# Autodesk Inventor assembly: Shoulder Joint Assembly
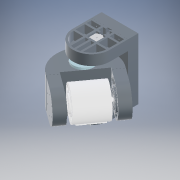
[picture p0: Inventor's stored thumbnail of the model, 180x180]
Saved by Autodesk Inventor 2017 SP1 (Build 210196100, 196)
## iProperties
Created: 2017-06-01
Part Number: Shoulder Joint Assembly
Document SubType Name: Assembly
Designer: Zach
Author: Zach
## Documents named in this file (15)
- C:\Users\Zach\Documents\GitHub\cr-laundry-robot\src\Body\Arm Assembly\Shoulder Joint Assembly\Shoulder Joint Assembly.iam
- C:\Users\Zach\Documents\GitHub\cr-laundry-robot\src\Body\Arm Assembly\Shoulder Joint Assembly\SJ002.ipt
- C:\Users\Zach\Documents\GitHub\cr-laundry-robot\src\Body\Arm Assembly\Shoulder Joint Assembly\SJ003.ipt
- C:\Users\Zach\Documents\GitHub\cr-laundry-robot\src\Body\Arm Assembly\Shoulder Joint Assembly\MC001.ipt
- C:\Users\Zach\Documents\GitHub\cr-laundry-robot\src\Body\Arm Assembly\Shoulder Joint Assembly\SJ001.ipt
- C:\Users\Zach\Documents\GitHub\cr-laundry-robot\src\Body\Arm Assembly\Shoulder Joint Assembly\MC002.ipt
- C:\Users\Zach\Documents\GitHub\cr-laundry-robot\lib\Stepper Motor - NEMA 17\NEMA17.ipt
- C:\Users\Zach\Documents\GitHub\cr-laundry-robot\src\Body\Arm Assembly\Shoulder Joint Assembly\SJ004.ipt
- C:\Users\Zach\Documents\GitHub\cr-laundry-robot\src\Body\Arm Assembly\Shoulder Joint Assembly\SJ005.ipt
- C:\Users\Zach\Documents\GitHub\cr-laundry-robot\src\Body\Arm Assembly\Shoulder Joint Assembly\SJ006.ipt
- C:\Users\Zach\Documents\GitHub\cr-laundry-robot\lib\U51105\U51105.ipt
- C:\Users\Zach\Documents\GitHub\cr-laundry-robot\lib\QS12MM250\QS12MM250.ipt
- C:\Users\Zach\Documents\GitHub\cr-laundry-robot\lib\6201RS\6201RS.ipt
- C:\Users\Zach\Documents\GitHub\cr-laundry-robot\src\Body\Arm Assembly\Shoulder Joint Assembly\SJ007.ipt
- C:\Users\Zach\Documents\GitHub\cr-laundry-robot\src\Body\Arm Assembly\Shoulder Joint Assembly\SJ008.ipt
## Components (29 placed, 14 different names)
1. MC001:1 — Mate:5, Mate:6, Mate:7, Mate:27, Mate:32
2. MC001:2 — Mate:41, Mate:42
3. SJ002:1 — Mate:1, Mate:4, Mate:5, Mate:6, Mate:7, Mate:8, Mate:9
4. SJ002:2 — Mate:18, Mate:19, Mate:20
5. SJ003:1 — Mate:1, Mate:4, Mate:8, Mate:9, Mate:18, Mate:19, Mate:20, Mate:71, Mate:72, Mate:73
6. SJ001:1 — Mate:23, Mate:24, Mate:25, Mate:43, Mate:44, Mate:47, Mate:48, Mate:49
7. MC002:1 — Mate:23, Mate:24, Mate:25, Mate:27, Mate:28, Mate:29, Mate:30, Mate:31
8. NEMA17:1 — Mate:28, Mate:29, Mate:30, Mate:31, Mate:32
9. SJ001:2 — Mate:37, Mate:38, Mate:39, Mate:43, Mate:45, Mate:46
10. MC002:2 — Mate:33, Mate:35, Mate:37, Mate:38, Mate:39, Mate:40, Mate:41
11. NEMA17:2 — Mate:33, Mate:35, Mate:40, Mate:42
12. SJ004:1 — Mate:44, Mate:45, Mate:46, Mate:57, Mate:58, Mate:59
13. SJ004:2 — Mate:47, Mate:48, Mate:49, Mate:54, Mate:55, Mate:56
14. SJ005:1 — Mate:54, Mate:55, Mate:56, Mate:60, Mate:63, Mate:65, Mate:66, Mate:67, Mate:69, Mate:70, Mate:80
15. SJ005:2 — Mate:57, Mate:58, Mate:59, Mate:64, Mate:68, Mate:82, Mate:84
16. SJ006:1 — Mate:63, Mate:64, Mate:65, Mate:66, Mate:75, Mate:76, Mate:81
17. SJ006:2 — Mate:67, Mate:68, Mate:69, Mate:70, Mate:78, Mate:79, Mate:83
18. NEMA17:3 — Mate:71, Mate:72, Mate:73
19. U51105:1 — Mate:75, Mate:76, Mate:90
20. U51105:2 — Mate:78, Mate:79, Mate:92
21. QS12MM250:1 — Mate:80, Mate:105, Mate:117, Mate:119, Mate:120
22. 6201RS:1 — Mate:81, Mate:82
23. 6201RS:2 — Mate:83, Mate:84
24. SJ007:1 — Mate:121, Mate:122, Mate:123, Mate:128
25. SJ008:1 — Mate:92, Mate:100, Mate:101, Mate:102, Mate:119, Mate:125, Mate:126, Mate:127
26. SJ008:2 — Mate:90, Mate:97, Mate:98, Mate:99, Mate:105, Mate:112, Mate:117, Mate:120, Mate:121, Mate:122, Mate:123, Mate:124
27. NEMA17:4 — Mate:97, Mate:98, Mate:99
28. NEMA17:5 — Mate:100, Mate:101, Mate:102
29. SJ007:2 — Mate:125, Mate:126, Mate:127, Mate:128
## Relationships (85: Mate 85)
- Mate:1: SJ002:1 ↔ SJ003:1
- Mate:4: SJ002:1 ↔ SJ003:1
- Mate:5: MC001:1 ↔ SJ002:1
- Mate:6: MC001:1 ↔ SJ002:1
- Mate:7: MC001:1 ↔ SJ002:1
- Mate:8: SJ002:1 ↔ SJ003:1
- Mate:9: SJ002:1 ↔ SJ003:1
- [Mate]: MC001:2 ↔ SJ002:2
- [Mate]: MC001:2 ↔ SJ002:2
- [Mate]: MC001:2 ↔ SJ002:2
- Mate:18: SJ002:2 ↔ SJ003:1
- Mate:19: SJ002:2 ↔ SJ003:1
- Mate:20: SJ002:2 ↔ SJ003:1
- Mate:23: SJ001:1 ↔ MC002:1
- Mate:24: SJ001:1 ↔ MC002:1
- Mate:25: SJ001:1 ↔ MC002:1
- Mate:27: MC001:1 ↔ MC002:1
- Mate:28: MC002:1 ↔ NEMA17:1
- Mate:29: MC002:1 ↔ NEMA17:1
- Mate:30: MC002:1 ↔ NEMA17:1
- Mate:31: MC002:1 ↔ NEMA17:1
- Mate:32: MC001:1 ↔ NEMA17:1
- Mate:33: MC002:2 ↔ NEMA17:2
- Mate:35: MC002:2 ↔ NEMA17:2
- Mate:37: SJ001:2 ↔ MC002:2
- Mate:38: SJ001:2 ↔ MC002:2
- Mate:39: SJ001:2 ↔ MC002:2
- Mate:40: MC002:2 ↔ NEMA17:2
- Mate:41: MC001:2 ↔ MC002:2
- Mate:42: MC001:2 ↔ NEMA17:2
- Mate:43: SJ001:1 ↔ SJ001:2
- Mate:44: SJ001:1 ↔ SJ004:1
- Mate:45: SJ001:2 ↔ SJ004:1
- Mate:46: SJ001:2 ↔ SJ004:1
- Mate:47: SJ001:1 ↔ SJ004:2
- Mate:48: SJ001:1 ↔ SJ004:2
- Mate:49: SJ001:1 ↔ SJ004:2
- Mate:54: SJ004:2 ↔ SJ005:1
- Mate:55: SJ004:2 ↔ SJ005:1
- Mate:56: SJ004:2 ↔ SJ005:1
- Mate:57: SJ004:1 ↔ SJ005:2
- Mate:58: SJ004:1 ↔ SJ005:2
- Mate:59: SJ004:1 ↔ SJ005:2
- Mate:60: SJ005:1
- Mate:63: SJ005:1 ↔ SJ006:1
- Mate:64: SJ005:2 ↔ SJ006:1
- Mate:65: SJ005:1 ↔ SJ006:1
- Mate:66: SJ005:1 ↔ SJ006:1
- Mate:67: SJ005:1 ↔ SJ006:2
- Mate:68: SJ005:2 ↔ SJ006:2
- Mate:69: SJ005:1 ↔ SJ006:2
- Mate:70: SJ005:1 ↔ SJ006:2
- Mate:71: SJ003:1 ↔ NEMA17:3
- Mate:72: SJ003:1 ↔ NEMA17:3
- Mate:73: SJ003:1 ↔ NEMA17:3
- Mate:75: SJ006:1 ↔ U51105:1
- Mate:76: SJ006:1 ↔ U51105:1
- Mate:78: SJ006:2 ↔ U51105:2
- Mate:79: SJ006:2 ↔ U51105:2
- Mate:80: SJ005:1 ↔ QS12MM250:1
- Mate:81: SJ006:1 ↔ 6201RS:1
- Mate:82: SJ005:2 ↔ 6201RS:1
- Mate:83: SJ006:2 ↔ 6201RS:2
- Mate:84: SJ005:2 ↔ 6201RS:2
- Mate:90: U51105:1 ↔ SJ008:2
- Mate:92: U51105:2 ↔ SJ008:1
- Mate:97: SJ008:2 ↔ NEMA17:4
- Mate:98: SJ008:2 ↔ NEMA17:4
- Mate:99: SJ008:2 ↔ NEMA17:4
- Mate:100: SJ008:1 ↔ NEMA17:5
- Mate:101: SJ008:1 ↔ NEMA17:5
- Mate:102: SJ008:1 ↔ NEMA17:5
- Mate:105: QS12MM250:1 ↔ SJ008:2
- Mate:112: SJ008:2
- Mate:117: QS12MM250:1 ↔ SJ008:2
- Mate:119: QS12MM250:1 ↔ SJ008:1
- Mate:120: QS12MM250:1 ↔ SJ008:2
- Mate:121: SJ007:1 ↔ SJ008:2
- Mate:122: SJ007:1 ↔ SJ008:2
- Mate:123: SJ007:1 ↔ SJ008:2
- Mate:124: SJ008:2
- Mate:125: SJ008:1 ↔ SJ007:2
- Mate:126: SJ008:1 ↔ SJ007:2
- Mate:127: SJ008:1 ↔ SJ007:2
- Mate:128: SJ007:1 ↔ SJ007:2
## Named parameters: d15_d4 = 0 mm, d16_d5 = 0 mm, d17_d7 = 0 mm
